# Autodesk Inventor assembly: P00173-09-001
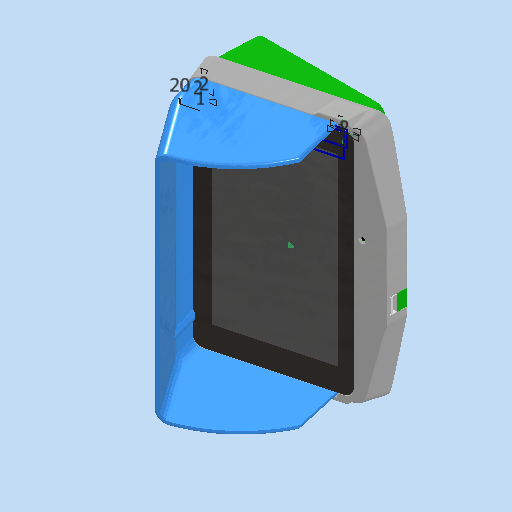
[picture p0: Inventor's stored thumbnail of the model, 512x512]
Saved by Autodesk Inventor 2022 (Build 260153070, 153G)
## iProperties
Created: 2021-03-30
Part Number: P00173-09-001
Document SubType Name: Assembly
Designer: MPM
Description: PAPER WALLET TERMINAL
Author: MPM
Comments: M2-Paypad 3d files for a Cardano blockchain payment terminal. Copyright (C) 2021 Maarten Menheere This program is free software; you can redistribute it and/or modify it under the terms of the GNU General Public License as published by the Free Software Foundation; either version 2 of the License, or (at your option) any later version. This program is distributed in the hope that it will be useful, but WITHOUT ANY WARRANTY; without even the implied warranty of MERCHANTABILITY or FITNESS FOR A PARTICULAR PURPOSE.  See the GNU General Public License for more details. You should have received a copy of the GNU General Public License along with this program; if not, write to the Free Software Foundation, Inc., 51 Franklin Street, Fifth Floor, Boston, MA  02110-1301, USA.
## Documents named in this file (10)
- M:\M2tec\M2tec\P00173 Cashgenic\P00173-09 Paypad - PU Rubber\P00173-09-001.iam
- M:\M2tec\M2tec\P00173 Cashgenic\3D Drawing\PA03591_A - RASPBERRY PI 7_ TOUCHSCREEN.ipt
- M:\M2tec\M2tec\P00173 Cashgenic\P00173-09 Paypad - PU Rubber\P00173-09-002.ipt
- M:\M2tec\M2tec\P00173 Cashgenic\P00173-09 Paypad - PU Rubber\P00173-09-004.ipt
- M:\M2tec\M2tec\P00173 Cashgenic\P00173-09 Paypad - PU Rubber\P00173-09-005.ipt
- M:\M2tec\M2tec\P00173 Cashgenic\P00173-02 Terminal met printer\raspberry-pi-camera-module-v2-1.snapshot.3\RspCameraMia.iam
- M:\M2tec\M2tec\P00173 Cashgenic\P00173-09 Paypad - PU Rubber\P00173-09-008.ipt
- M:\M2tec\M2tec\P00173 Cashgenic\P00173-08 Paypad - Spuitgiet\Raspberry-Pi-4-Model-B-03.ipt
- M:\M2tec\M2tec\P00173 Cashgenic\P00173-09 Paypad - PU Rubber\P00173-09-010.ipt
- M:\M2tec\M2tec\P00173 Cashgenic\P00173-09 Paypad - PU Rubber\P00173-09-013.ipt
## Components (9 placed, 9 different names)
1. PA03591_A - RASPBERRY PI 7_ TOUCHSCREEN:1 — Mate:8, Mate:22
2. P00173-09-002:1
3. P00173-09-010:1 — Mate:22
4. P00173-09-004:1 — Mate:18, Mate:19, Mate:20
5. P00173-09-005:1
6. RspCameraMia:1 [sub-assembly]
7. P00173-09-008:2 — Flush:1, Flush:2, Flush:3
8. Raspberry-Pi-4-Model-B-03:1 — Mate:18, Mate:19, Mate:20
9. P00173-09-013:1
## Relationships (8: Mate 5, Flush 3)
- Mate:8: PA03591_A - RASPBERRY PI 7_ TOUCHSCREEN:1
- Mate:18: P00173-09-004:1 ↔ Raspberry-Pi-4-Model-B-03:1
- Mate:19: P00173-09-004:1 ↔ Raspberry-Pi-4-Model-B-03:1
- Mate:20: P00173-09-004:1 ↔ Raspberry-Pi-4-Model-B-03:1
- Flush:1: P00173-09-008:2
- Flush:2: P00173-09-008:2
- Flush:3: P00173-09-008:2
- Mate:22 (0.25 mm): PA03591_A - RASPBERRY PI 7_ TOUCHSCREEN:1 ↔ P00173-09-010:1
